# Autodesk Inventor assembly: Excavator_complete
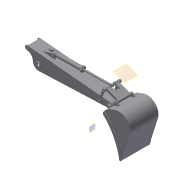
[picture p0: Inventor's stored thumbnail of the model, 180x180]
Saved by Autodesk Inventor 2022 (Build 260148000, 148)
## iProperties
Created: 2005-12-13
Part Number: Excavator_complete
Document SubType Name: Assembly
Designer: dchu
Translation Standard: IGES 5.3
File Name: Excavator.igs
Preprocessor: IBM CATIA IGES - CATIA Version 5 Release 14
Postprocessor: Build: 211m, Release: 10 - Date: Fri 03/18/2005
Sent Units: MM
Uncertainty: 0.001
Author: dchu
## Documents named in this file (9)
- C:\Autodesk Inventor 2022 Advanced Assembly Modeling Practice Files\Inventor Studio - Excavator\Excavator_complete.iam
- C:\Autodesk Inventor 2022 Advanced Assembly Modeling Practice Files\Inventor Studio - Excavator\SubfigureDefinition.ipt
- C:\Autodesk Inventor 2022 Advanced Assembly Modeling Practice Files\Inventor Studio - Excavator\SubfigureDefinitionA.ipt
- C:\Autodesk Inventor 2022 Advanced Assembly Modeling Practice Files\Inventor Studio - Excavator\SubfigureDefinitionB.ipt
- C:\Autodesk Inventor 2022 Advanced Assembly Modeling Practice Files\Inventor Studio - Excavator\SubfigureDefinition.iam
- C:\Autodesk Inventor 2022 Advanced Assembly Modeling Practice Files\Inventor Studio - Excavator\SubfigureDefinitionE.ipt
- C:\Autodesk Inventor 2022 Advanced Assembly Modeling Practice Files\Inventor Studio - Excavator\SubfigureDefinitionF.ipt
- C:\Autodesk Inventor 2022 Advanced Assembly Modeling Practice Files\Inventor Studio - Excavator\SubfigureDefinitionG.ipt
- C:\Autodesk Inventor 2022 Advanced Assembly Modeling Practice Files\Inventor Studio - Excavator\Bucket.ipt
## Components (9 placed, 8 different names)
1. ExcavatorArm — Mate:1, Mate:2, Mate:6, Mate:7, Mate:8, Mate:9, Mate:15, Mate:16, Mate:18
2. CylinderTube — Mate:1, Mate:2, Mate:3, Mate:4, Mate:5
3. CylinderStop — Mate:4, Mate:5, Mate:20
4. Cylinder [sub-assembly] — Mate:3, Mate:14, Mate:20
5. SubfigureDefinition:1
6. Link:1 — Mate:8, Mate:9, Mate:12, Mate:13
7. Link:2 — Mate:6, Mate:7, Mate:10, Mate:11
8. Linkage — Mate:10, Mate:11, Mate:12, Mate:13, Mate:14, Mate:17, Mate:19
9. Bucket:1 — Mate:15, Mate:16, Mate:17, Mate:18, Mate:19
## Relationships (20: Mate 20)
- Mate:1: ExcavatorArm ↔ CylinderTube
- Mate:2: ExcavatorArm ↔ CylinderTube
- Mate:3: CylinderTube ↔ Cylinder
- Mate:4: CylinderTube ↔ CylinderStop
- Mate:5: CylinderTube ↔ CylinderStop
- Mate:6: ExcavatorArm ↔ Link:2
- Mate:7: ExcavatorArm ↔ Link:2
- Mate:8: ExcavatorArm ↔ Link:1
- Mate:9: ExcavatorArm ↔ Link:1
- Mate:10: Link:2 ↔ Linkage
- Mate:11: Link:2 ↔ Linkage
- Mate:12: Link:1 ↔ Linkage
- Mate:13: Link:1 ↔ Linkage
- Mate:14: Cylinder ↔ Linkage
- Mate:15: ExcavatorArm ↔ Bucket:1
- Mate:16: ExcavatorArm ↔ Bucket:1
- Mate:17: Linkage ↔ Bucket:1
- Mate:18: ExcavatorArm ↔ Bucket:1
- Mate:19: Linkage ↔ Bucket:1
- Mate:20 (500 mm): CylinderStop ↔ Cylinder
